# Autodesk Inventor assembly: Сборка3
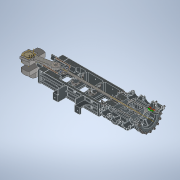
[picture p0: Inventor's stored thumbnail of the model, 180x180]
Saved by Autodesk Inventor 2021 (Build 250183000, 183)
## iProperties
Created: 2020-11-22
Part Number: Сборка3
Document SubType Name: Assembly
Designer: Тимоха
Author: Тимоха
## Documents named in this file (58)
- C:\Users\Тимоха\Desktop\КР Компрессор\compressor\Сборка3.iam
- C:\Users\Тимоха\Desktop\КР Компрессор\compressor\Верхняя часть поршня.ipt
- C:\Users\Тимоха\Desktop\КР Компрессор\compressor\Втулка.ipt
- C:\Users\Тимоха\Desktop\КР Компрессор\compressor\Гайка шток-поршень.ipt
- C:\Users\Тимоха\Desktop\КР Компрессор\compressor\Дроссельное кольцо.ipt
- C:\Users\Тимоха\Desktop\КР Компрессор\compressor\Клапан1.iam
- C:\Users\Тимоха\Desktop\КР Компрессор\compressor\Кольцо поршень-шток верх.ipt
- C:\Users\Тимоха\Desktop\КР Компрессор\compressor\Кольцо поршень-шток низ.ipt
- C:\Users\Тимоха\Desktop\КР Компрессор\compressor\Кольцо поршня.ipt
- C:\Users\Тимоха\Desktop\КР Компрессор\compressor\Кольцо сальника.ipt
- C:\Users\Тимоха\Desktop\КР Компрессор\compressor\Корпус дросселя.ipt
- C:\Users\Тимоха\Desktop\КР Компрессор\compressor\Корпус сальника.ipt
- C:\Users\Тимоха\Desktop\КР Компрессор\compressor\Крышка сальников.ipt
- C:\Users\Тимоха\Desktop\КР Компрессор\compressor\Крышка стакана.ipt
- C:\Users\Тимоха\Desktop\КР Компрессор\compressor\Крышка цилиндра 1.ipt
- C:\Users\Тимоха\Desktop\КР Компрессор\compressor\Крышка цилиндра 2.ipt
- C:\Users\Тимоха\Desktop\КР Компрессор\compressor\Нижняя часть поршня.ipt
- C:\Users\Тимоха\Desktop\КР Компрессор\compressor\Опорное кольцо.ipt
- C:\Users\Тимоха\Desktop\КР Компрессор\compressor\Прокладка клапана.ipt
- C:\Users\Тимоха\Desktop\КР Компрессор\compressor\Пружина дросселя.ipt
- C:\Users\Тимоха\Desktop\КР Компрессор\compressor\Пружина сальника.ipt
- C:\Users\Тимоха\Desktop\КР Компрессор\compressor\Стакан1.ipt
- C:\Users\Тимоха\Desktop\КР Компрессор\compressor\Цилиндр2.ipt
- C:\Users\Тимоха\Desktop\КР Компрессор\compressor\Шток.ipt
- C:\Users\Тимоха\Documents\Inventor\Content Center Files\R2021\ru-RU\Stud GOST 22034-76\Шпилька M20-6g×50 ГОСТ 22034-76.ipt
- C:\Users\Тимоха\Documents\Inventor\Content Center Files\R2021\ru-RU\GOST 10450-78\Шайба 21 ГОСТ 10450-78.ipt
- C:\Users\Тимоха\Documents\Inventor\Content Center Files\R2021\ru-RU\GOST 15521-70\Гайка M20-6H ГОСТ 15521-70.ipt
- C:\Users\Тимоха\Documents\Inventor\Content Center Files\R2021\ru-RU\GOST 11371-78  A\Шайба 24 ГОСТ 11371-78.ipt
- C:\Users\Тимоха\Documents\Inventor\Content Center Files\R2021\ru-RU\Stud GOST 22038-76\Шпилька M24-6g×70 ГОСТ 22038-76.ipt
- C:\Users\Тимоха\Documents\Inventor\Content Center Files\R2021\ru-RU\Nut GOST 15524-70\Гайка M24-6H ГОСТ 15524-70.ipt
- C:\Users\Тимоха\Documents\Inventor\Content Center Files\R2021\ru-RU\Bolt GOST R 50274-92\Болт M8-6g×20-F ГОСТ Р 50274-92.ipt
- C:\Users\Тимоха\Desktop\КР Компрессор\compressor\Деталь5.ipt
- C:\Users\Тимоха\Desktop\КР Компрессор\compressor\Деталь6.ipt
- C:\Users\Тимоха\Desktop\КР Компрессор\compressor\Прокладка воды зад.ipt
- C:\Users\Тимоха\Desktop\КР Компрессор\compressor\Крышка воды зад.ipt
- C:\Users\Тимоха\Documents\Inventor\Content Center Files\R2021\ru-RU\GOST 15521-70\Гайка M10-6H ГОСТ 15521-70.ipt
- C:\Users\Тимоха\Documents\Inventor\Content Center Files\R2021\ru-RU\Stud GOST 22034-76\Шпилька M10-6g×45 ГОСТ 22034-76.ipt
- C:\Users\Тимоха\Documents\Inventor\Content Center Files\R2021\ru-RU\Washer GOST 9065-75\Шайба 12 ГОСТ 9065-75.ipt
- C:\Users\Тимоха\Desktop\КР Компрессор\compressor\Фонарь.ipt
- C:\Users\Тимоха\Documents\Inventor\Content Center Files\R2021\ru-RU\Stud GOST 22038-76\Шпилька M20-6g×80 ГОСТ 22038-76.ipt
- C:\Users\Тимоха\Documents\Inventor\Content Center Files\R2021\ru-RU\GOST 6402-70\Шайба  22 L ГОСТ 6402-70.ipt
- C:\Users\Тимоха\Documents\Inventor\Content Center Files\R2021\ru-RU\Nut GOST ISO 8673-2014\Копия Копия гайки M20x1,5-6H ГОСТ 5915-70.ipt
- C:\Users\Тимоха\Desktop\КР Компрессор\compressor\Корпус сальника перегородка 1.ipt
- C:\Users\Тимоха\Desktop\КР Компрессор\compressor\Крышка перегородки11.ipt
- C:\Users\Тимоха\Desktop\КР Компрессор\compressor\Крышка перегородки12.ipt
- C:\Users\Тимоха\Desktop\КР Компрессор\compressor\Придав перегородки1.ipt
- C:\Users\Тимоха\Desktop\КР Компрессор\compressor\Корпус маслосъемника.ipt
- C:\Users\Тимоха\Desktop\КР Компрессор\compressor\Крышка перегородки21.ipt
- C:\Users\Тимоха\Desktop\КР Компрессор\compressor\Крышка перегородки22.ipt
- C:\Users\Тимоха\Desktop\КР Компрессор\compressor\Маслосъемная пружина.ipt
- C:\Users\Тимоха\Desktop\КР Компрессор\compressor\Маслосъемное кольцо.ipt
- C:\Users\Тимоха\Documents\Inventor\Content Center Files\R2021\ru-RU\GOST 11738-84\Винт M10-6gx20 ГОСТ 11738-84.ipt
- C:\Users\Тимоха\Documents\Inventor\Content Center Files\R2021\ru-RU\GOST 11371-78  A\Шайба 12 ГОСТ 11371-78.ipt
- C:\Users\Тимоха\Documents\Inventor\Content Center Files\R2021\ru-RU\GOST 11738-84\Винт M10-6gx25 ГОСТ 11738-84.ipt
- C:\Users\Тимоха\Desktop\КР Компрессор\compressor\Крейцкопфф.iam
- C:\Users\Тимоха\Desktop\КР Компрессор\compressor\Вал.ipt
- C:\Users\Тимоха\Desktop\КР Компрессор\compressor\Крышка фонаря 1.ipt
- C:\Users\Тимоха\Desktop\КР Компрессор\compressor\Крышка фонаря 2.ipt
## Components (442 placed, 57 different names)
1. Втулка:1 — Жесткий:9, Жесткий:12
2. Дроссельное кольцо:1 — Жесткий:21, Жесткий:22
3. Клапан1:1 [sub-assembly] — Жесткий:11, С поворотом:4
4. Корпус дросселя:1 — Жесткий:22, С поворотом:6
5. Крышка сальников:1 — Жесткий:72, Жесткий:73, Жесткий:143
6. Крышка стакана:1 — С поворотом:5
7. Крышка цилиндра 1:1 — Жесткий:12, С поворотом:9, Жесткий:198, Угол:1, Угол:2, Угол:3
8. Крышка цилиндра 2:1 — Жесткий:13, С поворотом:6, Жесткий:79, Жесткий:142, Жесткий:145, С поворотом:16
9. Прокладка клапана:1 — Жесткий:10, Жесткий:11
10. Пружина дросселя:1 — Жесткий:21
11. Стакан1:1 — С поворотом:4, С поворотом:5
12. Цилиндр2:1 — Жесткий:9, Жесткий:10, Жесткий:13, Жесткий:74, Жесткий:76, Жесткий:80, Заподлицо:1, Заподлицо:2, Заподлицо:5, Заподлицо:6
13. Кольцо сальника:4
14. Корпус сальника:2 — Жесткий:65
15. Пружина сальника:4
16. Кольцо сальника:5
17. Пружина сальника:5
18. Кольцо сальника:6
19. Пружина сальника:6
20. Кольцо сальника:7
21. Корпус сальника:3 — Жесткий:69, Жесткий:73
22. Пружина сальника:7
23. Кольцо сальника:8
24. Пружина сальника:8
25. Кольцо сальника:9
26. Пружина сальника:9
27. Кольцо сальника:10
28. Корпус сальника:4 — Жесткий:66
29. Пружина сальника:10
30. Кольцо сальника:11
31. Пружина сальника:11
32. Кольцо сальника:12
33. Пружина сальника:12
34. Кольцо сальника:13
35. Корпус сальника:5 — Жесткий:68
36. Пружина сальника:13
37. Кольцо сальника:14
38. Пружина сальника:14
39. Кольцо сальника:15
40. Пружина сальника:15
41. Кольцо сальника:16
42. Корпус сальника:6 — Жесткий:68, Жесткий:69
43. Пружина сальника:16
44. Кольцо сальника:17
45. Пружина сальника:17
46. Кольцо сальника:18
47. Пружина сальника:18
48. Кольцо сальника:19
49. Корпус сальника:7 — Жесткий:65, Жесткий:66
50. Пружина сальника:19
51. Кольцо сальника:20
52. Пружина сальника:20
53. Кольцо сальника:21
54. Пружина сальника:21
55. Кольцо сальника:22 — Жесткий:70, Жесткий:140
56. Кольцо сальника:23 — Жесткий:70, Жесткий:71, Жесткий:139
57. Кольцо сальника:24 — Жесткий:71, Жесткий:72, Жесткий:141
58. Болт ГОСТ Р 50274-92 M8-6g×20-F:2 — Жесткий:82
59. Болт ГОСТ Р 50274-92 M8-6g×20-F:3 — Жесткий:81
60. Деталь5:1 — Заподлицо:1, Заподлицо:2, Заподлицо:3, Заподлицо:4
61. Деталь6:1 — Заподлицо:3, Заподлицо:4, Жесткий:81, Жесткий:82, С поворотом:10, С поворотом:11, С поворотом:12, С поворотом:13, С поворотом:14, Жесткий:83, Жесткий:84, Жесткий:85, Жесткий:86, Жесткий:87, Жесткий:88, Жесткий:89, Жесткий:90, Жесткий:91, Жесткий:92, Жесткий:93, Жесткий:94, Жесткий:95, Жесткий:96, Жесткий:97, Жесткий:98, Жесткий:99, Жесткий:100, Жесткий:101, Жесткий:102, Жесткий:103, Жесткий:104, Жесткий:105, Жесткий:106, Жесткий:107
62. Прокладка воды зад:1 — Заподлицо:5, Заподлицо:6, Заподлицо:7, Заподлицо:8
63. Крышка воды зад:1 — Заподлицо:7, Заподлицо:8, С поворотом:15, Жесткий:108, Жесткий:109, Жесткий:110, Жесткий:111, Жесткий:112, Жесткий:113, Жесткий:114, Жесткий:115, Жесткий:116, Жесткий:117, Жесткий:118, Жесткий:119, Жесткий:120, Жесткий:121, Жесткий:122, Жесткий:123, Жесткий:124, Жесткий:125, Жесткий:126, Жесткий:127, Жесткий:128, Жесткий:129, Жесткий:130, Жесткий:131, Жесткий:132, Жесткий:133, Жесткий:134, Жесткий:135, Жесткий:136, Жесткий:137, Жесткий:138
64. Болт ГОСТ Р 50274-92 M8-6g×20-F:33 — С поворотом:14
65. Болт ГОСТ Р 50274-92 M8-6g×20-F:34 — Жесткий:85
66. Болт ГОСТ Р 50274-92 M8-6g×20-F:35 — С поворотом:11
67. Болт ГОСТ Р 50274-92 M8-6g×20-F:36 — С поворотом:10
68. Болт ГОСТ Р 50274-92 M8-6g×20-F:37 — Жесткий:83
69. Болт ГОСТ Р 50274-92 M8-6g×20-F:38 — Жесткий:84
70. Болт ГОСТ Р 50274-92 M8-6g×20-F:39 — С поворотом:12
71. Болт ГОСТ Р 50274-92 M8-6g×20-F:40 — С поворотом:13
72. Болт ГОСТ Р 50274-92 M8-6g×20-F:41 — Жесткий:91
73. Болт ГОСТ Р 50274-92 M8-6g×20-F:42 — Жесткий:90
74. Болт ГОСТ Р 50274-92 M8-6g×20-F:43 — Жесткий:87
75. Болт ГОСТ Р 50274-92 M8-6g×20-F:44 — Жесткий:86
76. Болт ГОСТ Р 50274-92 M8-6g×20-F:45 — Жесткий:89
77. Болт ГОСТ Р 50274-92 M8-6g×20-F:46 — Жесткий:93
78. Болт ГОСТ Р 50274-92 M8-6g×20-F:47 — Жесткий:88
79. Болт ГОСТ Р 50274-92 M8-6g×20-F:48 — Жесткий:92
80. Болт ГОСТ Р 50274-92 M8-6g×20-F:49 — Жесткий:99
81. Болт ГОСТ Р 50274-92 M8-6g×20-F:50 — Жесткий:98
82. Болт ГОСТ Р 50274-92 M8-6g×20-F:51 — Жесткий:97
83. Болт ГОСТ Р 50274-92 M8-6g×20-F:52 — Жесткий:94
84. Болт ГОСТ Р 50274-92 M8-6g×20-F:53 — Жесткий:95
85. Болт ГОСТ Р 50274-92 M8-6g×20-F:54 — Жесткий:102
86. Болт ГОСТ Р 50274-92 M8-6g×20-F:55 — Жесткий:100
87. Болт ГОСТ Р 50274-92 M8-6g×20-F:56 — Жесткий:101
88. Болт ГОСТ Р 50274-92 M8-6g×20-F:58 — Жесткий:106
89. Болт ГОСТ Р 50274-92 M8-6g×20-F:59 — Жесткий:104
90. Болт ГОСТ Р 50274-92 M8-6g×20-F:60 — Жесткий:96
91. Болт ГОСТ Р 50274-92 M8-6g×20-F:61 — Жесткий:107
92. Болт ГОСТ Р 50274-92 M8-6g×20-F:63 — Жесткий:103
93. Болт ГОСТ Р 50274-92 M8-6g×20-F:64 — Жесткий:105
94. Болт ГОСТ Р 50274-92 M8-6g×20-F:68 — С поворотом:15
95. Болт ГОСТ Р 50274-92 M8-6g×20-F:97 — Жесткий:108
96. Болт ГОСТ Р 50274-92 M8-6g×20-F:98 — Жесткий:110
97. Болт ГОСТ Р 50274-92 M8-6g×20-F:99 — Жесткий:109
98. Болт ГОСТ Р 50274-92 M8-6g×20-F:100 — Жесткий:111
99. Болт ГОСТ Р 50274-92 M8-6g×20-F:101 — Жесткий:113
100. Болт ГОСТ Р 50274-92 M8-6g×20-F:102 — Жесткий:112
101. Болт ГОСТ Р 50274-92 M8-6g×20-F:103 — Жесткий:114
102. Болт ГОСТ Р 50274-92 M8-6g×20-F:104 — Жесткий:115
103. Болт ГОСТ Р 50274-92 M8-6g×20-F:105 — Жесткий:116
104. Болт ГОСТ Р 50274-92 M8-6g×20-F:106 — Жесткий:118
105. Болт ГОСТ Р 50274-92 M8-6g×20-F:107 — Жесткий:130
106. Болт ГОСТ Р 50274-92 M8-6g×20-F:108 — Жесткий:134
107. Болт ГОСТ Р 50274-92 M8-6g×20-F:109 — Жесткий:133
108. Болт ГОСТ Р 50274-92 M8-6g×20-F:110 — Жесткий:131
109. Болт ГОСТ Р 50274-92 M8-6g×20-F:111 — Жесткий:135
110. Болт ГОСТ Р 50274-92 M8-6g×20-F:112 — Жесткий:132
111. Болт ГОСТ Р 50274-92 M8-6g×20-F:117 — Жесткий:117
112. Болт ГОСТ Р 50274-92 M8-6g×20-F:118 — Жесткий:119
113. Болт ГОСТ Р 50274-92 M8-6g×20-F:119 — Жесткий:120
114. Болт ГОСТ Р 50274-92 M8-6g×20-F:120 — Жесткий:121
115. Болт ГОСТ Р 50274-92 M8-6g×20-F:121 — Жесткий:122
116. Болт ГОСТ Р 50274-92 M8-6g×20-F:122 — Жесткий:123
117. Болт ГОСТ Р 50274-92 M8-6g×20-F:123 — Жесткий:124
118. Болт ГОСТ Р 50274-92 M8-6g×20-F:124 — Жесткий:125
119. Болт ГОСТ Р 50274-92 M8-6g×20-F:125 — Жесткий:126
120. Болт ГОСТ Р 50274-92 M8-6g×20-F:126 — Жесткий:127
121. Болт ГОСТ Р 50274-92 M8-6g×20-F:130 — Жесткий:129
122. Болт ГОСТ Р 50274-92 M8-6g×20-F:137 — Жесткий:128
123. Болт ГОСТ Р 50274-92 M8-6g×20-F:138 — Жесткий:137
124. Болт ГОСТ Р 50274-92 M8-6g×20-F:139 — Жесткий:136
125. Болт ГОСТ Р 50274-92 M8-6g×20-F:140 — Жесткий:138
126. Пружина сальника:22 — Жесткий:141
127. Пружина сальника:23 — Жесткий:140
128. Пружина сальника:24 — Жесткий:139
129. Фонарь:1 — Жесткий:145, Жесткий:146, Жесткий:160, Жесткий:168, Жесткий:189, Заподлицо:9, Заподлицо:10, Заподлицо:11, Заподлицо:12
130. Кольцо сальника:25 — Жесткий:148, Жесткий:152
131. Корпус сальника перегородка 1:1 — Жесткий:158, Жесткий:159, Жесткий:161, Жесткий:162
132. Крышка перегородки11:1 — Жесткий:160, Жесткий:161, Жесткий:163
133. Крышка перегородки12:1 — Жесткий:162, Жесткий:188
134. Придав перегородки1:1 — Жесткий:163, Жесткий:184
135. Пружина сальника:25 — Жесткий:148
136. Кольцо сальника:26 — Жесткий:151, Жесткий:158
137. Пружина сальника:26
138. Кольцо сальника:27 — Жесткий:151, Жесткий:152
139. Пружина сальника:27
140. Кольцо сальника:28 — Жесткий:159
141. Пружина сальника:28
142. Кольцо сальника:29
143. Пружина сальника:29
144. Кольцо сальника:30
145. Пружина сальника:30
146. Корпус маслосъемника:1 — Жесткий:167, Жесткий:175
147. Крышка перегородки21:1 — Жесткий:168, Жесткий:174, Жесткий:175, Жесткий:176, Жесткий:179
148. Крышка перегородки22:1 — Жесткий:176, Жесткий:185
149. Маслосъемное кольцо:1 — Жесткий:166, Жесткий:177
150. Придав перегородки1:2 — Жесткий:179, Жесткий:180
151. Маслосъемное кольцо:2 — Жесткий:166, Жесткий:167, Жесткий:178
152. Кольцо сальника:31 — Жесткий:174
153. Пружина сальника:31
154. Кольцо сальника:32
155. Пружина сальника:32
156. Кольцо сальника:33
157. Пружина сальника:33
158. Маслосъемная пружина:3 — Жесткий:177
159. Маслосъемная пружина:4 — Жесткий:178
160. Крейцкопфф:1 [sub-assembly] — Жесткий:189, Угол:1, Угол:2, Угол:3, С поворотом:19, Угол:4
161. Верхняя часть поршня:2 — Жесткий:198
162. Кольцо поршень-шток низ:2
163. Кольцо поршня:4
164. Нижняя часть поршня:2
165. Опорное кольцо:3
166. Кольцо поршня:5
167. Кольцо поршня:6
168. Опорное кольцо:4
169. Гайка шток-поршень:2
170. Кольцо поршень-шток верх:2
171. Шток:2
172. Вал:1 — С поворотом:19, Угол:4
173. Крышка фонаря 1:1 — Заподлицо:9, Заподлицо:10
174. Крышка фонаря 2:1 — Заподлицо:11, Заподлицо:12
175. Гайка ГОСТ 15524-70 M24:1 — Жесткий:77
176. Шайба  ГОСТ 11371-78 25:1 — Жесткий:77, С поворотом:9
177. Шпилька ГОСТ 22038-76 M24-6g×70:1 — Жесткий:76
178. Гайка ГОСТ 15524-70 M24:2
179. Шайба  ГОСТ 11371-78 25:2
180. Шпилька ГОСТ 22038-76 M24-6g×70:2
181. Гайка ГОСТ 15524-70 M24:3
182. Шайба  ГОСТ 11371-78 25:3
183. Шпилька ГОСТ 22038-76 M24-6g×70:3
184. Гайка ГОСТ 15524-70 M24:4
185. Шайба  ГОСТ 11371-78 25:4
186. Шпилька ГОСТ 22038-76 M24-6g×70:4
187. Гайка ГОСТ 15524-70 M24:5
188. Шайба  ГОСТ 11371-78 25:5
189. Шпилька ГОСТ 22038-76 M24-6g×70:5
190. Гайка ГОСТ 15524-70 M24:6
191. Шайба  ГОСТ 11371-78 25:6
192. Шпилька ГОСТ 22038-76 M24-6g×70:6
193. Гайка ГОСТ 15524-70 M24:7
194. Шайба  ГОСТ 11371-78 25:7
195. Шпилька ГОСТ 22038-76 M24-6g×70:7
196. Гайка ГОСТ 15524-70 M24:8
197. Шайба  ГОСТ 11371-78 25:8
198. Шпилька ГОСТ 22038-76 M24-6g×70:8
199. Гайка ГОСТ 15524-70 M24:9
200. Шайба  ГОСТ 11371-78 25:9
201. Шпилька ГОСТ 22038-76 M24-6g×70:9
202. Гайка ГОСТ 15524-70 M24:10
203. Шайба  ГОСТ 11371-78 25:10
204. Шпилька ГОСТ 22038-76 M24-6g×70:10
205. Гайка ГОСТ 15524-70 M24:11
206. Шайба  ГОСТ 11371-78 25:11
207. Шпилька ГОСТ 22038-76 M24-6g×70:11
208. Гайка ГОСТ 15524-70 M24:12
209. Шайба  ГОСТ 11371-78 25:12
210. Шпилька ГОСТ 22038-76 M24-6g×70:12
211. Гайка ГОСТ 15524-70 M24:13
212. Шайба  ГОСТ 11371-78 25:13
213. Шпилька ГОСТ 22038-76 M24-6g×70:13
214. Гайка ГОСТ 15524-70 M24:14
215. Шайба  ГОСТ 11371-78 25:14
216. Шпилька ГОСТ 22038-76 M24-6g×70:14
217. Гайка ГОСТ 15524-70 M24:15
218. Шайба  ГОСТ 11371-78 25:15
219. Шпилька ГОСТ 22038-76 M24-6g×70:15
220. Гайка ГОСТ 15524-70 M24:16
221. Шайба  ГОСТ 11371-78 25:16
222. Шпилька ГОСТ 22038-76 M24-6g×70:16
223. Шпилька ГОСТ 22038-76 M24-6g×70:17 — Жесткий:80
224. Гайка ГОСТ 15524-70 M24:17
225. Шайба  ГОСТ 11371-78 25:17 — Жесткий:79
226. Шпилька ГОСТ 22038-76 M24-6g×70:18
227. Гайка ГОСТ 15524-70 M24:18
228. Шайба  ГОСТ 11371-78 25:18
229. Шпилька ГОСТ 22038-76 M24-6g×70:19
230. Гайка ГОСТ 15524-70 M24:19
231. Шайба  ГОСТ 11371-78 25:19
232. Шпилька ГОСТ 22038-76 M24-6g×70:20
233. Гайка ГОСТ 15524-70 M24:20
234. Шайба  ГОСТ 11371-78 25:20
235. Шпилька ГОСТ 22038-76 M24-6g×70:21
236. Гайка ГОСТ 15524-70 M24:21
237. Шайба  ГОСТ 11371-78 25:21
238. Шпилька ГОСТ 22038-76 M24-6g×70:22
239. Гайка ГОСТ 15524-70 M24:22
240. Шайба  ГОСТ 11371-78 25:22
241. Шпилька ГОСТ 22038-76 M24-6g×70:23
242. Гайка ГОСТ 15524-70 M24:23
243. Шайба  ГОСТ 11371-78 25:23
244. Шпилька ГОСТ 22038-76 M24-6g×70:24
245. Гайка ГОСТ 15524-70 M24:24
246. Шайба  ГОСТ 11371-78 25:24
247. Шпилька ГОСТ 22038-76 M24-6g×70:25
248. Гайка ГОСТ 15524-70 M24:25
249. Шайба  ГОСТ 11371-78 25:25
250. Шпилька ГОСТ 22038-76 M24-6g×70:26
251. Гайка ГОСТ 15524-70 M24:26
252. Шайба  ГОСТ 11371-78 25:26
253. Шпилька ГОСТ 22038-76 M24-6g×70:27
254. Гайка ГОСТ 15524-70 M24:27
255. Шайба  ГОСТ 11371-78 25:27
256. Шпилька ГОСТ 22038-76 M24-6g×70:28
257. Гайка ГОСТ 15524-70 M24:28
258. Шайба  ГОСТ 11371-78 25:28
259. Шпилька ГОСТ 22038-76 M24-6g×70:29
260. Гайка ГОСТ 15524-70 M24:29
261. Шайба  ГОСТ 11371-78 25:29
262. Шпилька ГОСТ 22038-76 M24-6g×70:30
263. Гайка ГОСТ 15524-70 M24:30
264. Шайба  ГОСТ 11371-78 25:30
265. Шпилька ГОСТ 22038-76 M24-6g×70:31
266. Гайка ГОСТ 15524-70 M24:31
267. Шайба  ГОСТ 11371-78 25:31
268. Шпилька ГОСТ 22038-76 M24-6g×70:32
269. Гайка ГОСТ 15524-70 M24:32
270. Шайба  ГОСТ 11371-78 25:32
271. Шпилька ГОСТ 22034-76 M10-6g×45:1 — Жесткий:142
272. Гайка ГОСТ 15521-70 M10:1 — Жесткий:144
273. Шайба ГОСТ 9065-75 12:1 — Жесткий:143, Жесткий:144
274. Шпилька ГОСТ 22034-76 M10-6g×45:2
275. Гайка ГОСТ 15521-70 M10:2
276. Шайба ГОСТ 9065-75 12:2
277. Шпилька ГОСТ 22034-76 M10-6g×45:3
278. Гайка ГОСТ 15521-70 M10:3
279. Шайба ГОСТ 9065-75 12:3
280. Шпилька ГОСТ 22034-76 M10-6g×45:4
281. Гайка ГОСТ 15521-70 M10:4
282. Шайба ГОСТ 9065-75 12:4
283. Шпилька ГОСТ 22034-76 M10-6g×45:5
284. Гайка ГОСТ 15521-70 M10:5
285. Шайба ГОСТ 9065-75 12:5
286. Шпилька ГОСТ 22034-76 M10-6g×45:6
287. Гайка ГОСТ 15521-70 M10:6
288. Шайба ГОСТ 9065-75 12:6
289. Шпилька ГОСТ 22034-76 M10-6g×45:7
290. Гайка ГОСТ 15521-70 M10:7
291. Шайба ГОСТ 9065-75 12:7
292. Шпилька ГОСТ 22034-76 M10-6g×45:8
293. Гайка ГОСТ 15521-70 M10:8
294. Шайба ГОСТ 9065-75 12:8
295. Шпилька ГОСТ 22034-76 M10-6g×45:9
296. Гайка ГОСТ 15521-70 M10:9
297. Шайба ГОСТ 9065-75 12:9
298. Шпилька ГОСТ 22034-76 M10-6g×45:10
299. Гайка ГОСТ 15521-70 M10:10
300. Шайба ГОСТ 9065-75 12:10
301. Шпилька ГОСТ 22038-76 M20-6g×80:1 — С поворотом:16
302. Гайка ГОСТ ISO 8673-2014 M20x1,5:1 — Жесткий:147
303. Шайба ГОСТ 6402-70 22 L:1 — Жесткий:146, Жесткий:147
304. Шпилька ГОСТ 22038-76 M20-6g×80:2
305. Гайка ГОСТ ISO 8673-2014 M20x1,5:2
306. Шайба ГОСТ 6402-70 22 L:2
307. Шпилька ГОСТ 22038-76 M20-6g×80:3
308. Гайка ГОСТ ISO 8673-2014 M20x1,5:3
309. Шайба ГОСТ 6402-70 22 L:3
310. Шпилька ГОСТ 22038-76 M20-6g×80:4
311. Гайка ГОСТ ISO 8673-2014 M20x1,5:4
312. Шайба ГОСТ 6402-70 22 L:4
313. Шпилька ГОСТ 22038-76 M20-6g×80:5
314. Гайка ГОСТ ISO 8673-2014 M20x1,5:5
315. Шайба ГОСТ 6402-70 22 L:5
316. Шпилька ГОСТ 22038-76 M20-6g×80:6
317. Гайка ГОСТ ISO 8673-2014 M20x1,5:6
318. Шайба ГОСТ 6402-70 22 L:6
319. Шпилька ГОСТ 22038-76 M20-6g×80:7
320. Гайка ГОСТ ISO 8673-2014 M20x1,5:7
321. Шайба ГОСТ 6402-70 22 L:7
322. Шпилька ГОСТ 22038-76 M20-6g×80:8
323. Гайка ГОСТ ISO 8673-2014 M20x1,5:8
324. Шайба ГОСТ 6402-70 22 L:8
325. Шпилька ГОСТ 22038-76 M20-6g×80:9
326. Гайка ГОСТ ISO 8673-2014 M20x1,5:9
327. Шайба ГОСТ 6402-70 22 L:9
328. Шпилька ГОСТ 22038-76 M20-6g×80:10
329. Гайка ГОСТ ISO 8673-2014 M20x1,5:10
330. Шайба ГОСТ 6402-70 22 L:10
331. Шпилька ГОСТ 22038-76 M20-6g×80:11
332. Гайка ГОСТ ISO 8673-2014 M20x1,5:11
333. Шайба ГОСТ 6402-70 22 L:11
334. Шпилька ГОСТ 22038-76 M20-6g×80:12
335. Гайка ГОСТ ISO 8673-2014 M20x1,5:12
336. Шайба ГОСТ 6402-70 22 L:12
337. Шпилька ГОСТ 22038-76 M20-6g×80:13
338. Гайка ГОСТ ISO 8673-2014 M20x1,5:13
339. Шайба ГОСТ 6402-70 22 L:13
340. Шпилька ГОСТ 22038-76 M20-6g×80:14
341. Гайка ГОСТ ISO 8673-2014 M20x1,5:14
342. Шайба ГОСТ 6402-70 22 L:14
343. Шпилька ГОСТ 22038-76 M20-6g×80:15
344. Гайка ГОСТ ISO 8673-2014 M20x1,5:15
345. Шайба ГОСТ 6402-70 22 L:15
346. Шпилька ГОСТ 22038-76 M20-6g×80:16
347. Гайка ГОСТ ISO 8673-2014 M20x1,5:16
348. Шайба ГОСТ 6402-70 22 L:16
349. Гайка ГОСТ 15521-70 M20:1 — Жесткий:75
350. Шпилька ГОСТ 22034-76 M20-6g×50:1 — Жесткий:74, Жесткий:75
351. Шайба ГОСТ 10450-78 21:1
352. Гайка ГОСТ 15521-70 M20:2
353. Шпилька ГОСТ 22034-76 M20-6g×50:2
354. Шайба ГОСТ 10450-78 21:2
355. Гайка ГОСТ 15521-70 M20:3
356. Шпилька ГОСТ 22034-76 M20-6g×50:3
357. Шайба ГОСТ 10450-78 21:3
358. Гайка ГОСТ 15521-70 M20:4
359. Шпилька ГОСТ 22034-76 M20-6g×50:4
360. Шайба ГОСТ 10450-78 21:4
361. Гайка ГОСТ 15521-70 M20:5
362. Шпилька ГОСТ 22034-76 M20-6g×50:5
363. Шайба ГОСТ 10450-78 21:5
364. Гайка ГОСТ 15521-70 M20:6
365. Шпилька ГОСТ 22034-76 M20-6g×50:6
366. Шайба ГОСТ 10450-78 21:6
367. Гайка ГОСТ 15521-70 M20:7
368. Шпилька ГОСТ 22034-76 M20-6g×50:7
369. Шайба ГОСТ 10450-78 21:7
370. Гайка ГОСТ 15521-70 M20:8
371. Шпилька ГОСТ 22034-76 M20-6g×50:8
372. Шайба ГОСТ 10450-78 21:8
373. Гайка ГОСТ 15521-70 M20:9
374. Шпилька ГОСТ 22034-76 M20-6g×50:9
375. Шайба ГОСТ 10450-78 21:9
376. Гайка ГОСТ 15521-70 M20:10
377. Шпилька ГОСТ 22034-76 M20-6g×50:10
378. Шайба ГОСТ 10450-78 21:10
379. Винт ГОСТ 11738-84 M 10x20:1 — Жесткий:181
380. Шайба  ГОСТ 11371-78 13:1 — Жесткий:180, Жесткий:181
381. Винт ГОСТ 11738-84 M 10x20:4
382. Шайба  ГОСТ 11371-78 13:4
383. Винт ГОСТ 11738-84 M 10x20:5
384. Шайба  ГОСТ 11371-78 13:5
385. Винт ГОСТ 11738-84 M 10x20:6
386. Шайба  ГОСТ 11371-78 13:6
387. Винт ГОСТ 11738-84 M 10x20:7
388. Шайба  ГОСТ 11371-78 13:7
389. Винт ГОСТ 11738-84 M 10x20:8
390. Шайба  ГОСТ 11371-78 13:8
391. Винт ГОСТ 11738-84 M 10x20:9
392. Шайба  ГОСТ 11371-78 13:9
393. Винт ГОСТ 11738-84 M 10x20:10
394. Шайба  ГОСТ 11371-78 13:10
395. Винт ГОСТ 11738-84 M 10x20:3
396. Шайба  ГОСТ 11371-78 13:3 — Жесткий:184
397. Винт ГОСТ 11738-84 M 10x20:11
398. Шайба  ГОСТ 11371-78 13:11
399. Винт ГОСТ 11738-84 M 10x20:12
400. Шайба  ГОСТ 11371-78 13:12
401. Винт ГОСТ 11738-84 M 10x20:13
402. Шайба  ГОСТ 11371-78 13:13
403. Винт ГОСТ 11738-84 M 10x20:14
404. Шайба  ГОСТ 11371-78 13:14
405. Винт ГОСТ 11738-84 M 10x20:15
406. Шайба  ГОСТ 11371-78 13:15
407. Винт ГОСТ 11738-84 M 10x20:16
408. Шайба  ГОСТ 11371-78 13:16
409. Винт ГОСТ 11738-84 M 10x20:17
410. Шайба  ГОСТ 11371-78 13:17
411. Винт ГОСТ 11738-84 M 10x25:2
412. Шайба  ГОСТ 11371-78 13:19 — Жесткий:188
413. Винт ГОСТ 11738-84 M 10x25:3
414. Шайба  ГОСТ 11371-78 13:20
415. Винт ГОСТ 11738-84 M 10x25:4
416. Шайба  ГОСТ 11371-78 13:21
417. Винт ГОСТ 11738-84 M 10x25:5
418. Шайба  ГОСТ 11371-78 13:22
419. Винт ГОСТ 11738-84 M 10x25:6
420. Шайба  ГОСТ 11371-78 13:23
421. Винт ГОСТ 11738-84 M 10x25:7
422. Шайба  ГОСТ 11371-78 13:24
423. Винт ГОСТ 11738-84 M 10x25:8
424. Шайба  ГОСТ 11371-78 13:25
425. Винт ГОСТ 11738-84 M 10x25:9
426. Шайба  ГОСТ 11371-78 13:26
427. Шайба  ГОСТ 11371-78 13:18 — Жесткий:185, Жесткий:186
428. Винт ГОСТ 11738-84 M 10x25:1 — Жесткий:186
429. Шайба  ГОСТ 11371-78 13:27
430. Винт ГОСТ 11738-84 M 10x25:10
431. Шайба  ГОСТ 11371-78 13:28
432. Винт ГОСТ 11738-84 M 10x25:11
433. Шайба  ГОСТ 11371-78 13:29
434. Винт ГОСТ 11738-84 M 10x25:12
435. Шайба  ГОСТ 11371-78 13:30
436. Винт ГОСТ 11738-84 M 10x25:13
437. Шайба  ГОСТ 11371-78 13:31
438. Винт ГОСТ 11738-84 M 10x25:14
439. Шайба  ГОСТ 11371-78 13:32
440. Винт ГОСТ 11738-84 M 10x25:15
441. Шайба  ГОСТ 11371-78 13:33
442. Винт ГОСТ 11738-84 M 10x25:16
## Component patterns: (16 elements, first: Гайка ГОСТ 15524-70 M24:1 + Шайба  ГОСТ 11371-78 25:1 + Шпилька ГОСТ 22038-76 M24-6g×70:1), (16 elements, first: Шпилька ГОСТ 22038-76 M24-6g×70:17 + Гайка ГОСТ 15524-70 M24:17 + Шайба  ГОСТ 11371-78 25:17), (10 elements, first: Шпилька ГОСТ 22034-76 M10-6g×45:1 + Гайка ГОСТ 15521-70 M10:1 + Шайба ГОСТ 9065-75 12:1), (16 elements, first: Шпилька ГОСТ 22038-76 M20-6g×80:1 + Гайка ГОСТ ISO 8673-2014 M20x1,5:1 + Шайба ГОСТ 6402-70 22 L:1), (10 elements, first: Гайка ГОСТ 15521-70 M20:1 + Шпилька ГОСТ 22034-76 M20-6g×50:1 + Шайба ГОСТ 10450-78 21:1), (8 elements, first: Винт ГОСТ 11738-84 M 10x20:1 + Шайба  ГОСТ 11371-78 13:1), (8 elements, first: Винт ГОСТ 11738-84 M 10x20:3 + Шайба  ГОСТ 11371-78 13:3), (8 elements, first: Винт ГОСТ 11738-84 M 10x25:2 + Шайба  ГОСТ 11371-78 13:19), (8 elements, first: Шайба  ГОСТ 11371-78 13:18 + Винт ГОСТ 11738-84 M 10x25:1)
## Relationships (204: WeldJoint 173, RevoluteJoint 15, Flush 12, Angle 4)
- Жесткий:9 [WeldJoint]: Втулка:1 ↔ Цилиндр2:1
- Жесткий:10 [WeldJoint]: Прокладка клапана:1 ↔ Цилиндр2:1
- Жесткий:11 [WeldJoint]: Клапан1:1 ↔ Прокладка клапана:1
- С поворотом:4 [RevoluteJoint]: Клапан1:1 ↔ Стакан1:1
- С поворотом:5 [RevoluteJoint]: Крышка стакана:1 ↔ Стакан1:1
- Жесткий:12 [WeldJoint]: Втулка:1 ↔ Крышка цилиндра 1:1
- Жесткий:13 [WeldJoint]: Крышка цилиндра 2:1 ↔ Цилиндр2:1
- Жесткий:21 [WeldJoint] (2 mm): Дроссельное кольцо:1 ↔ Пружина дросселя:1
- Жесткий:22 [WeldJoint]: Дроссельное кольцо:1 ↔ Корпус дросселя:1
- С поворотом:6 [RevoluteJoint]: Корпус дросселя:1 ↔ Крышка цилиндра 2:1
- [WeldJoint] (-1 mm): Кольцо сальника:4 ↔ Пружина сальника:4
- [WeldJoint] (-1 mm): Кольцо сальника:5 ↔ Пружина сальника:5
- [WeldJoint] (-1 mm): Кольцо сальника:6 ↔ Пружина сальника:6
- [WeldJoint]: Кольцо сальника:5 ↔ Кольцо сальника:6
- [WeldJoint]: Кольцо сальника:4 ↔ Кольцо сальника:5
- [WeldJoint]: Корпус сальника:2 ↔ Кольцо сальника:6
- [WeldJoint] (-1 mm): Кольцо сальника:7 ↔ Пружина сальника:7
- [WeldJoint] (-1 mm): Кольцо сальника:8 ↔ Пружина сальника:8
- [WeldJoint] (-1 mm): Кольцо сальника:9 ↔ Пружина сальника:9
- [WeldJoint]: Кольцо сальника:8 ↔ Кольцо сальника:9
- [WeldJoint]: Кольцо сальника:7 ↔ Кольцо сальника:8
- [WeldJoint]: Корпус сальника:3 ↔ Кольцо сальника:9
- [WeldJoint] (-1 mm): Кольцо сальника:10 ↔ Пружина сальника:10
- [WeldJoint] (-1 mm): Кольцо сальника:11 ↔ Пружина сальника:11
- [WeldJoint] (-1 mm): Кольцо сальника:12 ↔ Пружина сальника:12
- [WeldJoint]: Кольцо сальника:11 ↔ Кольцо сальника:12
- [WeldJoint]: Кольцо сальника:10 ↔ Кольцо сальника:11
- [WeldJoint]: Корпус сальника:4 ↔ Кольцо сальника:12
- [WeldJoint] (-1 mm): Кольцо сальника:13 ↔ Пружина сальника:13
- [WeldJoint] (-1 mm): Кольцо сальника:14 ↔ Пружина сальника:14
- [WeldJoint] (-1 mm): Кольцо сальника:15 ↔ Пружина сальника:15
- [WeldJoint]: Кольцо сальника:14 ↔ Кольцо сальника:15
- [WeldJoint]: Кольцо сальника:13 ↔ Кольцо сальника:14
- [WeldJoint]: Корпус сальника:5 ↔ Кольцо сальника:15
- [WeldJoint] (-1 mm): Кольцо сальника:16 ↔ Пружина сальника:16
- [WeldJoint] (-1 mm): Кольцо сальника:17 ↔ Пружина сальника:17
- [WeldJoint] (-1 mm): Кольцо сальника:18 ↔ Пружина сальника:18
- [WeldJoint]: Кольцо сальника:17 ↔ Кольцо сальника:18
- [WeldJoint]: Кольцо сальника:16 ↔ Кольцо сальника:17
- [WeldJoint]: Корпус сальника:6 ↔ Кольцо сальника:18
- [WeldJoint] (-1 mm): Кольцо сальника:19 ↔ Пружина сальника:19
- [WeldJoint] (-1 mm): Кольцо сальника:20 ↔ Пружина сальника:20
- [WeldJoint] (-1 mm): Кольцо сальника:21 ↔ Пружина сальника:21
- [WeldJoint]: Кольцо сальника:20 ↔ Кольцо сальника:21
- [WeldJoint]: Кольцо сальника:19 ↔ Кольцо сальника:20
- [WeldJoint]: Корпус сальника:7 ↔ Кольцо сальника:21
- Жесткий:65 [WeldJoint]: Корпус сальника:2 ↔ Корпус сальника:7
- Жесткий:66 [WeldJoint]: Корпус сальника:4 ↔ Корпус сальника:7
- Жесткий:68 [WeldJoint]: Корпус сальника:5 ↔ Корпус сальника:6
- Жесткий:69 [WeldJoint]: Корпус сальника:3 ↔ Корпус сальника:6
- Жесткий:70 [WeldJoint]: Кольцо сальника:22 ↔ Кольцо сальника:23
- Жесткий:71 [WeldJoint]: Кольцо сальника:23 ↔ Кольцо сальника:24
- Жесткий:72 [WeldJoint]: Крышка сальников:1 ↔ Кольцо сальника:24
- Жесткий:73 [WeldJoint]: Крышка сальников:1 ↔ Корпус сальника:3
- [RevoluteJoint]: Гайка ГОСТ 15521-70 M20:1 ↔ Шайба ГОСТ 10450-78 21:1
- Жесткий:74 [WeldJoint] (23.5 mm): Цилиндр2:1 ↔ Шпилька ГОСТ 22034-76 M20-6g×50:1
- Жесткий:75 [WeldJoint] (-2.75 mm): Гайка ГОСТ 15521-70 M20:1 ↔ Шпилька ГОСТ 22034-76 M20-6g×50:1
- Жесткий:76 [WeldJoint]: Цилиндр2:1 ↔ Шпилька ГОСТ 22038-76 M24-6g×70:1
- Жесткий:77 [WeldJoint]: Гайка ГОСТ 15524-70 M24:1 ↔ Шайба  ГОСТ 11371-78 25:1
- С поворотом:9 [RevoluteJoint]: Крышка цилиндра 1:1 ↔ Шайба  ГОСТ 11371-78 25:1
- [WeldJoint]: Гайка ГОСТ 15524-70 M24:17 ↔ Шайба  ГОСТ 11371-78 25:17
- Жесткий:79 [WeldJoint]: Крышка цилиндра 2:1 ↔ Шайба  ГОСТ 11371-78 25:17
- Жесткий:80 [WeldJoint]: Цилиндр2:1 ↔ Шпилька ГОСТ 22038-76 M24-6g×70:17
- Заподлицо:1 [Flush]: Цилиндр2:1 ↔ Деталь5:1
- Заподлицо:2 [Flush]: Цилиндр2:1 ↔ Деталь5:1
- Заподлицо:3 [Flush]: Деталь5:1 ↔ Деталь6:1
- Заподлицо:4 [Flush]: Деталь5:1 ↔ Деталь6:1
- Заподлицо:5 [Flush]: Цилиндр2:1 ↔ Прокладка воды зад:1
- Заподлицо:6 [Flush]: Цилиндр2:1 ↔ Прокладка воды зад:1
- Заподлицо:7 [Flush]: Прокладка воды зад:1 ↔ Крышка воды зад:1
- Заподлицо:8 [Flush]: Прокладка воды зад:1 ↔ Крышка воды зад:1
- Жесткий:81 [WeldJoint]: Болт ГОСТ Р 50274-92 M8-6g×20-F:3 ↔ Деталь6:1
- Жесткий:82 [WeldJoint]: Болт ГОСТ Р 50274-92 M8-6g×20-F:2 ↔ Деталь6:1
- С поворотом:10 [RevoluteJoint]: Деталь6:1 ↔ Болт ГОСТ Р 50274-92 M8-6g×20-F:36
- С поворотом:11 [RevoluteJoint]: Деталь6:1 ↔ Болт ГОСТ Р 50274-92 M8-6g×20-F:35
- С поворотом:12 [RevoluteJoint]: Деталь6:1 ↔ Болт ГОСТ Р 50274-92 M8-6g×20-F:39
- С поворотом:13 [RevoluteJoint]: Деталь6:1 ↔ Болт ГОСТ Р 50274-92 M8-6g×20-F:40
- С поворотом:14 [RevoluteJoint]: Деталь6:1 ↔ Болт ГОСТ Р 50274-92 M8-6g×20-F:33
- Жесткий:83 [WeldJoint]: Деталь6:1 ↔ Болт ГОСТ Р 50274-92 M8-6g×20-F:37
- Жесткий:84 [WeldJoint]: Деталь6:1 ↔ Болт ГОСТ Р 50274-92 M8-6g×20-F:38
- Жесткий:85 [WeldJoint]: Деталь6:1 ↔ Болт ГОСТ Р 50274-92 M8-6g×20-F:34
- Жесткий:86 [WeldJoint]: Деталь6:1 ↔ Болт ГОСТ Р 50274-92 M8-6g×20-F:44
- Жесткий:87 [WeldJoint]: Деталь6:1 ↔ Болт ГОСТ Р 50274-92 M8-6g×20-F:43
- Жесткий:88 [WeldJoint]: Деталь6:1 ↔ Болт ГОСТ Р 50274-92 M8-6g×20-F:47
- Жесткий:89 [WeldJoint]: Деталь6:1 ↔ Болт ГОСТ Р 50274-92 M8-6g×20-F:45
- Жесткий:90 [WeldJoint]: Деталь6:1 ↔ Болт ГОСТ Р 50274-92 M8-6g×20-F:42
- Жесткий:91 [WeldJoint]: Деталь6:1 ↔ Болт ГОСТ Р 50274-92 M8-6g×20-F:41
- Жесткий:92 [WeldJoint]: Деталь6:1 ↔ Болт ГОСТ Р 50274-92 M8-6g×20-F:48
- Жесткий:93 [WeldJoint]: Деталь6:1 ↔ Болт ГОСТ Р 50274-92 M8-6g×20-F:46
- Жесткий:94 [WeldJoint]: Деталь6:1 ↔ Болт ГОСТ Р 50274-92 M8-6g×20-F:52
- Жесткий:95 [WeldJoint]: Деталь6:1 ↔ Болт ГОСТ Р 50274-92 M8-6g×20-F:53
- Жесткий:96 [WeldJoint]: Деталь6:1 ↔ Болт ГОСТ Р 50274-92 M8-6g×20-F:60
- Жесткий:97 [WeldJoint]: Деталь6:1 ↔ Болт ГОСТ Р 50274-92 M8-6g×20-F:51
- Жесткий:98 [WeldJoint]: Деталь6:1 ↔ Болт ГОСТ Р 50274-92 M8-6g×20-F:50
- Жесткий:99 [WeldJoint]: Деталь6:1 ↔ Болт ГОСТ Р 50274-92 M8-6g×20-F:49
- Жесткий:100 [WeldJoint]: Деталь6:1 ↔ Болт ГОСТ Р 50274-92 M8-6g×20-F:55
- Жесткий:101 [WeldJoint]: Деталь6:1 ↔ Болт ГОСТ Р 50274-92 M8-6g×20-F:56
- Жесткий:102 [WeldJoint]: Деталь6:1 ↔ Болт ГОСТ Р 50274-92 M8-6g×20-F:54
- Жесткий:103 [WeldJoint]: Деталь6:1 ↔ Болт ГОСТ Р 50274-92 M8-6g×20-F:63
- Жесткий:104 [WeldJoint]: Деталь6:1 ↔ Болт ГОСТ Р 50274-92 M8-6g×20-F:59
- Жесткий:105 [WeldJoint]: Деталь6:1 ↔ Болт ГОСТ Р 50274-92 M8-6g×20-F:64
- Жесткий:106 [WeldJoint]: Деталь6:1 ↔ Болт ГОСТ Р 50274-92 M8-6g×20-F:58
- Жесткий:107 [WeldJoint]: Деталь6:1 ↔ Болт ГОСТ Р 50274-92 M8-6g×20-F:61
- С поворотом:15 [RevoluteJoint]: Крышка воды зад:1 ↔ Болт ГОСТ Р 50274-92 M8-6g×20-F:68
- Жесткий:108 [WeldJoint]: Крышка воды зад:1 ↔ Болт ГОСТ Р 50274-92 M8-6g×20-F:97
- Жесткий:109 [WeldJoint]: Крышка воды зад:1 ↔ Болт ГОСТ Р 50274-92 M8-6g×20-F:99
- Жесткий:110 [WeldJoint]: Крышка воды зад:1 ↔ Болт ГОСТ Р 50274-92 M8-6g×20-F:98
- Жесткий:111 [WeldJoint]: Крышка воды зад:1 ↔ Болт ГОСТ Р 50274-92 M8-6g×20-F:100
- Жесткий:112 [WeldJoint]: Крышка воды зад:1 ↔ Болт ГОСТ Р 50274-92 M8-6g×20-F:102
- Жесткий:113 [WeldJoint]: Крышка воды зад:1 ↔ Болт ГОСТ Р 50274-92 M8-6g×20-F:101
- Жесткий:114 [WeldJoint]: Крышка воды зад:1 ↔ Болт ГОСТ Р 50274-92 M8-6g×20-F:103
- Жесткий:115 [WeldJoint]: Крышка воды зад:1 ↔ Болт ГОСТ Р 50274-92 M8-6g×20-F:104
- Жесткий:116 [WeldJoint]: Крышка воды зад:1 ↔ Болт ГОСТ Р 50274-92 M8-6g×20-F:105
- Жесткий:117 [WeldJoint]: Крышка воды зад:1 ↔ Болт ГОСТ Р 50274-92 M8-6g×20-F:117
- Жесткий:118 [WeldJoint]: Крышка воды зад:1 ↔ Болт ГОСТ Р 50274-92 M8-6g×20-F:106
- Жесткий:119 [WeldJoint]: Крышка воды зад:1 ↔ Болт ГОСТ Р 50274-92 M8-6g×20-F:118
- Жесткий:120 [WeldJoint]: Крышка воды зад:1 ↔ Болт ГОСТ Р 50274-92 M8-6g×20-F:119
- Жесткий:121 [WeldJoint]: Крышка воды зад:1 ↔ Болт ГОСТ Р 50274-92 M8-6g×20-F:120
- Жесткий:122 [WeldJoint]: Крышка воды зад:1 ↔ Болт ГОСТ Р 50274-92 M8-6g×20-F:121
- Жесткий:123 [WeldJoint]: Крышка воды зад:1 ↔ Болт ГОСТ Р 50274-92 M8-6g×20-F:122
- Жесткий:124 [WeldJoint]: Крышка воды зад:1 ↔ Болт ГОСТ Р 50274-92 M8-6g×20-F:123
- Жесткий:125 [WeldJoint]: Крышка воды зад:1 ↔ Болт ГОСТ Р 50274-92 M8-6g×20-F:124
- Жесткий:126 [WeldJoint]: Крышка воды зад:1 ↔ Болт ГОСТ Р 50274-92 M8-6g×20-F:125
- Жесткий:127 [WeldJoint]: Крышка воды зад:1 ↔ Болт ГОСТ Р 50274-92 M8-6g×20-F:126
- Жесткий:128 [WeldJoint]: Крышка воды зад:1 ↔ Болт ГОСТ Р 50274-92 M8-6g×20-F:137
- Жесткий:129 [WeldJoint]: Крышка воды зад:1 ↔ Болт ГОСТ Р 50274-92 M8-6g×20-F:130
- Жесткий:130 [WeldJoint]: Крышка воды зад:1 ↔ Болт ГОСТ Р 50274-92 M8-6g×20-F:107
- Жесткий:131 [WeldJoint]: Крышка воды зад:1 ↔ Болт ГОСТ Р 50274-92 M8-6g×20-F:110
- Жесткий:132 [WeldJoint]: Крышка воды зад:1 ↔ Болт ГОСТ Р 50274-92 M8-6g×20-F:112
- Жесткий:133 [WeldJoint]: Крышка воды зад:1 ↔ Болт ГОСТ Р 50274-92 M8-6g×20-F:109
- Жесткий:134 [WeldJoint]: Крышка воды зад:1 ↔ Болт ГОСТ Р 50274-92 M8-6g×20-F:108
- Жесткий:135 [WeldJoint]: Крышка воды зад:1 ↔ Болт ГОСТ Р 50274-92 M8-6g×20-F:111
- Жесткий:136 [WeldJoint]: Крышка воды зад:1 ↔ Болт ГОСТ Р 50274-92 M8-6g×20-F:139
- Жесткий:137 [WeldJoint]: Крышка воды зад:1 ↔ Болт ГОСТ Р 50274-92 M8-6g×20-F:138
- Жесткий:138 [WeldJoint]: Крышка воды зад:1 ↔ Болт ГОСТ Р 50274-92 M8-6g×20-F:140
- Жесткий:139 [WeldJoint] (1 mm): Кольцо сальника:23 ↔ Пружина сальника:24
- Жесткий:140 [WeldJoint]: Кольцо сальника:22 ↔ Пружина сальника:23
- Жесткий:141 [WeldJoint]: Кольцо сальника:24 ↔ Пружина сальника:22
- Жесткий:142 [WeldJoint]: Крышка цилиндра 2:1 ↔ Шпилька ГОСТ 22034-76 M10-6g×45:1
- Жесткий:143 [WeldJoint]: Крышка сальников:1 ↔ Шайба ГОСТ 9065-75 12:1
- Жесткий:144 [WeldJoint]: Гайка ГОСТ 15521-70 M10:1 ↔ Шайба ГОСТ 9065-75 12:1
- Жесткий:145 [WeldJoint]: Крышка цилиндра 2:1 ↔ Фонарь:1
- С поворотом:16 [RevoluteJoint]: Крышка цилиндра 2:1 ↔ Шпилька ГОСТ 22038-76 M20-6g×80:1
- Жесткий:146 [WeldJoint]: Фонарь:1 ↔ Шайба ГОСТ 6402-70 22 L:1
- Жесткий:147 [WeldJoint]: Гайка ГОСТ ISO 8673-2014 M20x1,5:1 ↔ Шайба ГОСТ 6402-70 22 L:1
- Жесткий:148 [WeldJoint]: Кольцо сальника:25 ↔ Пружина сальника:25
- [WeldJoint]: Кольцо сальника:26 ↔ Пружина сальника:26
- [WeldJoint]: Кольцо сальника:27 ↔ Пружина сальника:27
- Жесткий:151 [WeldJoint]: Кольцо сальника:26 ↔ Кольцо сальника:27
- Жесткий:152 [WeldJoint]: Кольцо сальника:25 ↔ Кольцо сальника:27
- [WeldJoint]: Кольцо сальника:28 ↔ Пружина сальника:28
- [WeldJoint]: Кольцо сальника:29 ↔ Пружина сальника:29
- [WeldJoint]: Кольцо сальника:30 ↔ Пружина сальника:30
- [WeldJoint]: Кольцо сальника:29 ↔ Кольцо сальника:30
- [WeldJoint]: Кольцо сальника:28 ↔ Кольцо сальника:30
- Жесткий:158 [WeldJoint]: Корпус сальника перегородка 1:1 ↔ Кольцо сальника:26
- Жесткий:159 [WeldJoint]: Корпус сальника перегородка 1:1 ↔ Кольцо сальника:28
- Жесткий:160 [WeldJoint]: Фонарь:1 ↔ Крышка перегородки11:1
- Жесткий:161 [WeldJoint]: Корпус сальника перегородка 1:1 ↔ Крышка перегородки11:1
- Жесткий:162 [WeldJoint]: Корпус сальника перегородка 1:1 ↔ Крышка перегородки12:1
- Жесткий:163 [WeldJoint]: Крышка перегородки11:1 ↔ Придав перегородки1:1
- Жесткий:166 [WeldJoint]: Маслосъемное кольцо:1 ↔ Маслосъемное кольцо:2
- Жесткий:167 [WeldJoint]: Корпус маслосъемника:1 ↔ Маслосъемное кольцо:2
- Жесткий:168 [WeldJoint]: Фонарь:1 ↔ Крышка перегородки21:1
- [WeldJoint]: Кольцо сальника:31 ↔ Пружина сальника:31
- [WeldJoint]: Кольцо сальника:32 ↔ Пружина сальника:32
- [WeldJoint]: Кольцо сальника:33 ↔ Пружина сальника:33
- [WeldJoint]: Кольцо сальника:32 ↔ Кольцо сальника:33
- [WeldJoint]: Кольцо сальника:31 ↔ Кольцо сальника:33
- Жесткий:174 [WeldJoint]: Крышка перегородки21:1 ↔ Кольцо сальника:31
- Жесткий:175 [WeldJoint]: Корпус маслосъемника:1 ↔ Крышка перегородки21:1
- Жесткий:176 [WeldJoint]: Крышка перегородки21:1 ↔ Крышка перегородки22:1
- Жесткий:177 [WeldJoint]: Маслосъемное кольцо:1 ↔ Маслосъемная пружина:3
- Жесткий:178 [WeldJoint] (1 mm): Маслосъемное кольцо:2 ↔ Маслосъемная пружина:4
- Жесткий:179 [WeldJoint]: Крышка перегородки21:1 ↔ Придав перегородки1:2
- Жесткий:180 [WeldJoint]: Придав перегородки1:2 ↔ Шайба  ГОСТ 11371-78 13:1
- Жесткий:181 [WeldJoint]: Винт ГОСТ 11738-84 M 10x20:1 ↔ Шайба  ГОСТ 11371-78 13:1
- [WeldJoint]: Винт ГОСТ 11738-84 M 10x20:3 ↔ Шайба  ГОСТ 11371-78 13:3
- Жесткий:184 [WeldJoint]: Придав перегородки1:1 ↔ Шайба  ГОСТ 11371-78 13:3
- Жесткий:185 [WeldJoint]: Крышка перегородки22:1 ↔ Шайба  ГОСТ 11371-78 13:18
- Жесткий:186 [WeldJoint]: Шайба  ГОСТ 11371-78 13:18 ↔ Винт ГОСТ 11738-84 M 10x25:1
- [WeldJoint]: Винт ГОСТ 11738-84 M 10x25:2 ↔ Шайба  ГОСТ 11371-78 13:19
- Жесткий:188 [WeldJoint]: Крышка перегородки12:1 ↔ Шайба  ГОСТ 11371-78 13:19
- Жесткий:189 [WeldJoint]: Фонарь:1 ↔ Крейцкопфф:1
- [RevoluteJoint]: Верхняя часть поршня:2 ↔ Нижняя часть поршня:2
- [RevoluteJoint]: Верхняя часть поршня:2 ↔ Кольцо поршня:4
- [WeldJoint]: Нижняя часть поршня:2 ↔ Кольцо поршня:5
- [WeldJoint]: Нижняя часть поршня:2 ↔ Кольцо поршня:6
- [WeldJoint]: Верхняя часть поршня:2 ↔ Опорное кольцо:4
- [WeldJoint]: Нижняя часть поршня:2 ↔ Опорное кольцо:3
- [WeldJoint]: Кольцо поршень-шток низ:2 ↔ Нижняя часть поршня:2
- [WeldJoint]: Верхняя часть поршня:2 ↔ Кольцо поршень-шток верх:2
- [WeldJoint]: Гайка шток-поршень:2 ↔ Кольцо поршень-шток верх:2
- [WeldJoint]: Гайка шток-поршень:2 ↔ Шток:2
- Жесткий:198 [WeldJoint] (115 mm): Крышка цилиндра 1:1 ↔ Верхняя часть поршня:2
- Угол:1 [Angle] (45 deg): Крышка цилиндра 1:1 ↔ Крейцкопфф:1
- Угол:2 [Angle] (45 deg): Крышка цилиндра 1:1 ↔ Крейцкопфф:1
- Угол:3 [Angle] (45 deg): Крышка цилиндра 1:1 ↔ Крейцкопфф:1
- С поворотом:19 [RevoluteJoint]: Крейцкопфф:1 ↔ Вал:1
- Угол:4 [Angle] (0 deg): Крейцкопфф:1 ↔ Вал:1
- Заподлицо:9 [Flush]: Фонарь:1 ↔ Крышка фонаря 1:1
- Заподлицо:10 [Flush]: Фонарь:1 ↔ Крышка фонаря 1:1
- Заподлицо:11 [Flush]: Фонарь:1 ↔ Крышка фонаря 2:1
- Заподлицо:12 [Flush]: Фонарь:1 ↔ Крышка фонаря 2:1
## Named parameters: d45_d35 = -1 mm, d46_d36_d35 = -1 mm, d47_d37_d35 = -1 mm, d48_d38 = 0 mm, d49_d39 = 0 mm, d50_d40 = 0 mm, d53_d45_d35 = -1 mm, d54_d46_d36_d35 = -1 mm, d55_d47_d37_d35 = -1 mm, d56_d48_d38 = 0 mm, d57_d49_d39 = 0 mm, d58_d50_d40 = 0 mm, d60_d45_d35 = -1 mm, d61_d46_d36_d35 = -1 mm, d62_d47_d37_d35 = -1 mm, d63_d48_d38 = 0 mm, d64_d49_d39 = 0 mm, d65_d50_d40 = 0 mm, d67_d45_d35 = -1 mm, d68_d46_d36_d35 = -1 mm, d69_d47_d37_d35 = -1 mm, d70_d48_d38 = 0 mm, d71_d49_d39 = 0 mm, d72_d50_d40 = 0 mm, d74_d45_d35 = -1 mm, d75_d46_d36_d35 = -1 mm, d76_d47_d37_d35 = -1 mm, d77_d48_d38 = 0 mm, d78_d49_d39 = 0 mm, d79_d50_d40 = 0 mm, d81_d45_d35 = -1 mm, d82_d46_d36_d35 = -1 mm, d83_d47_d37_d35 = -1 mm, d84_d48_d38 = 0 mm, d85_d49_d39 = 0 mm, d86_d50_d40 = 0 mm, d101_d20 = 0 mm, d102_d21 = 30 deg, d114_d109 = 0 mm, d228_d227 = 0 mm, d229_d227 = 0 mm, d232_d227 = 0 mm, d233_d228_d227 = 0 mm, d234_d229_d227 = 0 mm, d235_d230 = 0 mm, d236_d231 = 0 mm, d248_d232_d227 = 0 mm, d249_d233_d228_d227 = 0 mm, d250_d234_d229_d227 = 0 mm, d251_d235_d230 = 0 mm, d252_d236_d231 = 0 mm, d262_d260 = 0 mm, d270_d269 = 0 mm, d278_d3 = 0 mm, d279_d4 = 105 deg, d280_d5 = 0 mm, d281_d6 = -75 deg, d282_d7 = 0 mm, d283_d8 = 0 mm, d284_d9 = 0 mm, d285_d10 = 0 mm, d286_d12 = 0 mm, d287_d20 = 0 mm, d288_d21 = 0 mm, d289_d22 = 0 mm
